# Autodesk Inventor assembly: 15102898-16-A-0200
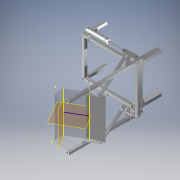
[picture p0: Inventor's stored thumbnail of the model, 180x180]
Saved by Autodesk Inventor 2017 (Build 210142000, 142)
## iProperties
Created: 2016-09-26
Part Number: 15102898-16-A-0200
Document SubType Name: Assembly
Designer: gus
Mass: 7782.67 g
Surface Area: 18020.1 cm^2
Volume: 2883.8 cm^3
Density: 2.69875 g/cm^3
Author: gus
## Documents named in this file (27)
- \\Mac\Home\Desktop\bunnybots 2016\15102898-16-Bunnybot-CAD\Bunnybot-To_be_renamed\15102898-16-A-0000\15102898-16-A-0200\15102898-16-A-0200.iam
- \\Mac\Home\Desktop\bunnybots 2016\15102898-16-Bunnybot-CAD\Bunnybot-To_be_renamed\15102898-16-A-0000\15102898-16-A-0200\15102898-16-P-0201.ipt
- \\Mac\Home\Desktop\bunnybots 2016\15102898-16-Bunnybot-CAD\Bunnybot-To_be_renamed\15102898-16-A-0000\15102898-16-A-0200\Imported Components\217-2732.20121205.ipt
- \\Mac\Home\Desktop\bunnybots 2016\15102898-16-Bunnybot-CAD\Bunnybot-To_be_renamed\15102898-16-A-0000\15102898-16-A-0200\15102898-16-P-0201_MIR.ipt
- \\Mac\Home\Desktop\bunnybots 2016\15102898-16-Bunnybot-CAD\Bunnybot-To_be_renamed\15102898-16-A-0000\15102898-16-A-0200\Imported Components\217-2732.20121205_MIR.ipt
- \\Mac\Home\Desktop\bunnybots 2016\15102898-16-Bunnybot-CAD\Bunnybot-To_be_renamed\15102898-16-A-0000\15102898-16-A-0200\15102898-16-P-0203.ipt
- \\Mac\Home\Desktop\bunnybots 2016\15102898-16-Bunnybot-CAD\Bunnybot-To_be_renamed\15102898-16-A-0000\15102898-16-A-0200\15102898-16-A-0205.ipt
- \\Mac\Home\Desktop\bunnybots 2016\15102898-16-Bunnybot-CAD\Bunnybot-To_be_renamed\15102898-16-A-0000\15102898-16-A-0200\AIS2015\175-DPEE5(F,D-231-1).iam
- \\Mac\Home\Desktop\bunnybots 2016\15102898-16-Bunnybot-CAD\Bunnybot-To_be_renamed\15102898-16-A-0000\15102898-16-A-0200\15102898-16-A-0204.iam
- \\Mac\Home\Desktop\bunnybots 2016\15102898-16-Bunnybot-CAD\Bunnybot-To_be_renamed\15102898-16-A-0000\15102898-16-A-0200\15102898-16-P-0205.ipt
- \\Mac\Home\Desktop\bunnybots 2016\15102898-16-Bunnybot-CAD\Bunnybot-To_be_renamed\15102898-16-A-0000\15102898-16-A-0200\Imported Components\91257A636_HIGH-STRENGTH GRADE 8 STEEL CAP SCREW.ipt
- \\Mac\Home\Desktop\bunnybots 2016\15102898-16-Bunnybot-CAD\Bunnybot-To_be_renamed\15102898-16-A-0000\15102898-16-A-0200\Imported Components\97135A230_GRADE 8 STEEL NYLON-INSERT LOCKNUT.ipt
- \\Mac\Home\Desktop\bunnybots 2016\15102898-16-Bunnybot-CAD\Bunnybot-To_be_renamed\15102898-16-A-0000\15102898-16-A-0200\15102898-16-P-0206.ipt
- \\Mac\Home\Desktop\bunnybots 2016\15102898-16-Bunnybot-CAD\Bunnybot-To_be_renamed\15102898-16-A-0000\15102898-16-A-0200\15102898-16-P-0207.ipt
- \\Mac\Home\Desktop\bunnybots 2016\15102898-16-Bunnybot-CAD\Bunnybot-To_be_renamed\15102898-16-A-0000\15102898-16-A-0200\15102898-16-P-0208.ipt
- \\Mac\Home\Desktop\bunnybots 2016\15102898-16-Bunnybot-CAD\Bunnybot-To_be_renamed\15102898-16-A-0000\15102898-16-A-0200\15102898-16-P-0209.ipt
- \\Mac\Home\Desktop\bunnybots 2016\15102898-16-Bunnybot-CAD\Bunnybot-To_be_renamed\15102898-16-A-0000\15102898-16-A-0200\15102898-16-P-0210.ipt
- \\Mac\Home\Desktop\bunnybots 2016\15102898-16-Bunnybot-CAD\Bunnybot-To_be_renamed\15102898-16-A-0000\15102898-16-A-0200\15102898-16-P-0211.ipt
- \\Mac\Home\Desktop\bunnybots 2016\15102898-16-Bunnybot-CAD\Bunnybot-To_be_renamed\15102898-16-A-0000\15102898-16-A-0200\15102898-16-P-0212.ipt
- \\Mac\Home\Desktop\bunnybots 2016\15102898-16-Bunnybot-CAD\Bunnybot-To_be_renamed\15102898-16-A-0000\15102898-16-A-0200\15102898-16-P-0213.ipt
- \\Mac\Home\Desktop\bunnybots 2016\15102898-16-Bunnybot-CAD\Bunnybot-To_be_renamed\15102898-16-A-0000\15102898-16-A-0200\15102898-16-P-0214.ipt
- \\Mac\Home\Desktop\bunnybots 2016\15102898-16-Bunnybot-CAD\Bunnybot-To_be_renamed\15102898-16-A-0000\15102898-16-A-0200\15102898-16-P-0215.ipt
- \\Mac\Home\Desktop\bunnybots 2016\15102898-16-Bunnybot-CAD\Bunnybot-To_be_renamed\15102898-16-A-0000\15102898-16-A-0200\15102898-16-P-0216.ipt
- \\Mac\Home\Desktop\bunnybots 2016\15102898-16-Bunnybot-CAD\Bunnybot-To_be_renamed\15102898-16-A-0000\15102898-16-A-0200\15102898-16-P-0217.ipt
- \\Mac\Home\Desktop\bunnybots 2016\15102898-16-Bunnybot-CAD\Bunnybot-To_be_renamed\15102898-16-A-0000\15102898-16-A-0200\15102898-16-P-0218.ipt
- \\Mac\Home\Desktop\bunnybots 2016\15102898-16-Bunnybot-CAD\Bunnybot-To_be_renamed\15102898-16-A-0000\15102898-16-A-0200\Imported Components\1556A170_BRACKET.ipt
- \\Mac\Home\Desktop\bunnybots 2016\15102898-16-Bunnybot-CAD\Bunnybot-To_be_renamed\15102898-16-A-0000\15102898-16-A-0200\15102898-16-P-0205_CPY.ipt
## Components (51 placed, 26 different names)
1. 15102898-16-P-0201:1 — Mate:1, Mate:4, Mate:5, Flush:9, Flush:10, Mate:14, Mate:32, Mate:42, Flush:34, Flush:35, Flush:36, Flush:56, Mate:83, Flush:91, Mate:86, Flush:94
2. 217-2732.20121205:1 — Mate:1, Mate:4, Mate:5, Cylindrical:6, Mate:22
3. 15102898-16-P-0201_MIR:1 — Flush:3, Mate:6, Mate:8, Flush:24, Mate:31, Mate:41, Flush:33, Flush:37, Mate:64, Mate:81, Flush:90, Mate:85, Flush:92, Flush:93
4. 217-2732.20121205_MIR:1 — Flush:3, Mate:6, Mate:8, Cylindrical:7, Mate:27
5. 15102898-16-P-0203:1 — Cylindrical:5, Mate:17, Mate:20, Mate:21, Cylindrical:6, Flush:40, Mate:47, Flush:59, Flush:61
6. 15102898-16-A-0205:1 — Flush:9, Flush:10, Mate:14, Mate:16, Flush:22, Flush:23, Flush:53, Flush:54, Flush:83, Flush:86, Mate:74, Flush:87, Mate:75
7. 175-DPEE5(F,D-231-1):1 [sub-assembly] — Mate:16, Cylindrical:4
8. 15102898-16-A-0204:1 [sub-assembly] — Cylindrical:4, Cylindrical:5, Mate:17
9. 15102898-16-P-0205:1 — Cylindrical:12, Mate:33, Mate:34, Mate:37, Flush:41, Mate:51, Mate:56, Flush:60
10. 15102898-16-P-0205:2 — Flush:21, Mate:26, Mate:27, Flush:42
11. 15102898-16-P-0205:3 — Flush:21, Cylindrical:13, Mate:30, Flush:51, Flush:71, Mate:62
12. 15102898-16-P-0205:4 — Mate:20, Mate:21, Mate:22, Flush:40, Flush:41
13. 15102898-16-P-0203:2 — Cylindrical:7, Mate:26, Cylindrical:9, Mate:29, Flush:42, Flush:51
14. 15102898-16-A-0205:2 — Flush:22, Flush:23, Flush:24, Flush:52, Flush:77, Mate:67, Flush:88, Mate:77, Mate:79, Flush:89
15. 175-DPEE5(F,D-231-1):2 [sub-assembly]
16. 15102898-16-A-0204:2 [sub-assembly] — Cylindrical:9, Mate:29
17. 91257A636_HIGH-STRENGTH GRADE 8 STEEL CAP SCREW:1 — Cylindrical:10, Cylindrical:13, Mate:30
18. 91257A636_HIGH-STRENGTH GRADE 8 STEEL CAP SCREW:2 — Cylindrical:11, Cylindrical:12, Mate:33, Mate:47
19. 97135A230_GRADE 8 STEEL NYLON-INSERT LOCKNUT:1 — Cylindrical:10, Mate:31
20. 97135A230_GRADE 8 STEEL NYLON-INSERT LOCKNUT:2 — Cylindrical:11, Mate:32
21. 15102898-16-P-0206:1 — Mate:34, Mate:35, Flush:27, Flush:28, Mate:36, Mate:38, Flush:31, Mate:39, Flush:63, Flush:69
22. 15102898-16-P-0207:1 — Mate:35, Flush:27, Flush:68, Flush:69
23. 15102898-16-P-0207:2 — Flush:28, Mate:36, Mate:37, Mate:51
24. 15102898-16-P-0208:1 — Mate:38, Flush:31, Flush:62, Flush:63
25. 15102898-16-P-0208:2 — Mate:39, Flush:70, Mate:60
26. 15102898-16-P-0209:1 — Mate:41, Flush:33, Mate:42, Flush:34, Mate:43, Mate:44, Mate:45
27. 15102898-16-P-0210:1 — Flush:35, Flush:36, Mate:43
28. 15102898-16-P-0210:2 — Mate:44, Flush:37, Mate:45
29. 15102898-16-P-0211:1 — Flush:52, Flush:53, Flush:54, Mate:52, Flush:55, Flush:76, Mate:68, Mate:71, Mate:73, Mate:84, Flush:95
30. 15102898-16-P-0212:1 — Mate:52, Flush:55, Cylindrical:16, Flush:56, Mate:54, Flush:81
31. 15102898-16-P-0213:1 — Cylindrical:15, Mate:55, Flush:57, Flush:58, Mate:57, Mate:58
32. 15102898-16-P-0214:1 — Cylindrical:15, Cylindrical:16, Mate:54, Mate:58, Flush:78, Flush:79
33. 15102898-16-P-0215:1 — Mate:55, Flush:57, Flush:58, Mate:63, Flush:74, Flush:75
34. 15102898-16-P-0216:1 — Flush:59, Mate:56, Flush:60, Flush:61, Flush:62, Mate:57, Flush:66, Flush:67, Flush:72, Mate:61
35. 15102898-16-P-0216:2 — Flush:66, Flush:67, Flush:68, Flush:70, Mate:60, Flush:71, Flush:73, Mate:62
36. 15102898-16-P-0217:1 — Flush:72, Mate:61, Flush:73
37. 15102898-16-P-0213:2 — Mate:63, Flush:74, Flush:75
38. 15102898-16-P-0214:2 — Flush:78, Flush:79, Mate:66
39. 15102898-16-P-0212:2 — Mate:65, Flush:80, Flush:81, Mate:66
40. 15102898-16-P-0211:2 — Flush:76, Mate:64, Flush:77, Mate:65, Flush:80, Flush:82, Mate:70, Mate:78, Mate:82
41. 15102898-16-P-0218:1 — Flush:82, Mate:67, Mate:68, Flush:83, Flush:84, Mate:69, Flush:85, Mate:72, Mate:76, Mate:80
42. 1556A170_BRACKET:1 — Flush:84, Mate:69, Mate:70
43. 1556A170_BRACKET:2 — Flush:85, Mate:71, Mate:72
44. 1556A170_BRACKET:3 — Flush:86, Mate:73, Mate:74
45. 1556A170_BRACKET:4 — Flush:87, Mate:75, Mate:76
46. 1556A170_BRACKET:5 — Flush:88, Mate:77, Mate:78
47. 1556A170_BRACKET:6 — Mate:79, Flush:89, Mate:80
48. 1556A170_BRACKET:7 — Mate:81, Mate:82, Flush:90
49. 1556A170_BRACKET:8 — Mate:83, Mate:84, Flush:91
50. 15102898-16-P-0205_CPY:1 — Mate:85, Flush:92, Flush:93
51. 15102898-16-P-0205_CPY:2 — Mate:86, Flush:94, Flush:95
## Relationships (138: Mate 65, Flush 61, CylindricalJoint 12)
- Mate:1: 15102898-16-P-0201:1 ↔ 217-2732.20121205:1
- Mate:4: 15102898-16-P-0201:1 ↔ 217-2732.20121205:1
- Mate:5: 15102898-16-P-0201:1 ↔ 217-2732.20121205:1
- Flush:3: 15102898-16-P-0201_MIR:1 ↔ 217-2732.20121205_MIR:1
- Mate:6: 15102898-16-P-0201_MIR:1 ↔ 217-2732.20121205_MIR:1
- Mate:8: 15102898-16-P-0201_MIR:1 ↔ 217-2732.20121205_MIR:1
- Flush:9: 15102898-16-P-0201:1 ↔ 15102898-16-A-0205:1
- Flush:10: 15102898-16-P-0201:1 ↔ 15102898-16-A-0205:1
- Mate:14 (467.995 mm): 15102898-16-P-0201:1 ↔ 15102898-16-A-0205:1
- Mate:16: 15102898-16-A-0205:1 ↔ 175-DPEE5(F,D-231-1):1
- Cylindrical:4: 175-DPEE5(F,D-231-1):1 ↔ 15102898-16-A-0204:1
- Cylindrical:5: 15102898-16-P-0203:1 ↔ 15102898-16-A-0204:1
- Mate:17: 15102898-16-P-0203:1 ↔ 15102898-16-A-0204:1
- Mate:20: 15102898-16-P-0203:1 ↔ 15102898-16-P-0205:4
- Mate:21: 15102898-16-P-0203:1 ↔ 15102898-16-P-0205:4
- Cylindrical:6: 217-2732.20121205:1 ↔ 15102898-16-P-0203:1
- Mate:22 (6.35 mm): 217-2732.20121205:1 ↔ 15102898-16-P-0205:4
- Flush:21: 15102898-16-P-0205:2 ↔ 15102898-16-P-0205:3
- Cylindrical:7: 217-2732.20121205_MIR:1 ↔ 15102898-16-P-0203:2
- Mate:26: 15102898-16-P-0205:2 ↔ 15102898-16-P-0203:2
- Mate:27 (6.35 mm): 217-2732.20121205_MIR:1 ↔ 15102898-16-P-0205:2
- [Mate]: 15102898-16-A-0205:2 ↔ 175-DPEE5(F,D-231-1):2
- [CylindricalJoint]: 175-DPEE5(F,D-231-1):2 ↔ 15102898-16-A-0204:2
- Flush:22: 15102898-16-A-0205:1 ↔ 15102898-16-A-0205:2
- Flush:23: 15102898-16-A-0205:1 ↔ 15102898-16-A-0205:2
- Flush:24: 15102898-16-P-0201_MIR:1 ↔ 15102898-16-A-0205:2
- Cylindrical:9: 15102898-16-P-0203:2 ↔ 15102898-16-A-0204:2
- Mate:29: 15102898-16-P-0203:2 ↔ 15102898-16-A-0204:2
- Cylindrical:10: 91257A636_HIGH-STRENGTH GRADE 8 STEEL CAP SCREW:1 ↔ 97135A230_GRADE 8 STEEL NYLON-INSERT LOCKNUT:1
- Cylindrical:11: 91257A636_HIGH-STRENGTH GRADE 8 STEEL CAP SCREW:2 ↔ 97135A230_GRADE 8 STEEL NYLON-INSERT LOCKNUT:2
- Cylindrical:12: 15102898-16-P-0205:1 ↔ 91257A636_HIGH-STRENGTH GRADE 8 STEEL CAP SCREW:2
- Cylindrical:13: 15102898-16-P-0205:3 ↔ 91257A636_HIGH-STRENGTH GRADE 8 STEEL CAP SCREW:1
- Mate:30: 15102898-16-P-0205:3 ↔ 91257A636_HIGH-STRENGTH GRADE 8 STEEL CAP SCREW:1
- Mate:31: 15102898-16-P-0201_MIR:1 ↔ 97135A230_GRADE 8 STEEL NYLON-INSERT LOCKNUT:1
- Mate:32: 15102898-16-P-0201:1 ↔ 97135A230_GRADE 8 STEEL NYLON-INSERT LOCKNUT:2
- Mate:33: 15102898-16-P-0205:1 ↔ 91257A636_HIGH-STRENGTH GRADE 8 STEEL CAP SCREW:2
- Mate:34: 15102898-16-P-0205:1 ↔ 15102898-16-P-0206:1
- Mate:35: 15102898-16-P-0206:1 ↔ 15102898-16-P-0207:1
- Flush:27: 15102898-16-P-0206:1 ↔ 15102898-16-P-0207:1
- Flush:28: 15102898-16-P-0206:1 ↔ 15102898-16-P-0207:2
- Mate:36: 15102898-16-P-0206:1 ↔ 15102898-16-P-0207:2
- Mate:37: 15102898-16-P-0205:1 ↔ 15102898-16-P-0207:2
- Mate:38: 15102898-16-P-0206:1 ↔ 15102898-16-P-0208:1
- Flush:31: 15102898-16-P-0206:1 ↔ 15102898-16-P-0208:1
- Mate:39: 15102898-16-P-0206:1 ↔ 15102898-16-P-0208:2
- Mate:41: 15102898-16-P-0201_MIR:1 ↔ 15102898-16-P-0209:1
- Flush:33: 15102898-16-P-0201_MIR:1 ↔ 15102898-16-P-0209:1
- Mate:42: 15102898-16-P-0201:1 ↔ 15102898-16-P-0209:1
- Flush:34 (38.1 mm): 15102898-16-P-0201:1 ↔ 15102898-16-P-0209:1
- Flush:35: 15102898-16-P-0201:1 ↔ 15102898-16-P-0210:1
- Flush:36: 15102898-16-P-0201:1 ↔ 15102898-16-P-0210:1
- Mate:43: 15102898-16-P-0209:1 ↔ 15102898-16-P-0210:1
- Mate:44: 15102898-16-P-0209:1 ↔ 15102898-16-P-0210:2
- Flush:37: 15102898-16-P-0201_MIR:1 ↔ 15102898-16-P-0210:2
- Mate:45: 15102898-16-P-0209:1 ↔ 15102898-16-P-0210:2
- Flush:40: 15102898-16-P-0203:1 ↔ 15102898-16-P-0205:4
- Mate:47: 15102898-16-P-0203:1 ↔ 91257A636_HIGH-STRENGTH GRADE 8 STEEL CAP SCREW:2
- Flush:41: 15102898-16-P-0205:1 ↔ 15102898-16-P-0205:4
- Flush:42: 15102898-16-P-0205:2 ↔ 15102898-16-P-0203:2
- Flush:51: 15102898-16-P-0205:3 ↔ 15102898-16-P-0203:2
- Mate:51: 15102898-16-P-0205:1 ↔ 15102898-16-P-0207:2
- Flush:52: 15102898-16-A-0205:2 ↔ 15102898-16-P-0211:1
- Flush:53: 15102898-16-A-0205:1 ↔ 15102898-16-P-0211:1
- Flush:54: 15102898-16-A-0205:1 ↔ 15102898-16-P-0211:1
- Mate:52: 15102898-16-P-0211:1 ↔ 15102898-16-P-0212:1
- Flush:55: 15102898-16-P-0211:1 ↔ 15102898-16-P-0212:1
- Cylindrical:15: 15102898-16-P-0213:1 ↔ 15102898-16-P-0214:1
- Cylindrical:16: 15102898-16-P-0212:1 ↔ 15102898-16-P-0214:1
- Flush:56 (105.7148 mm): 15102898-16-P-0201:1 ↔ 15102898-16-P-0212:1
- Mate:54: 15102898-16-P-0212:1 ↔ 15102898-16-P-0214:1
- Mate:55: 15102898-16-P-0213:1 ↔ 15102898-16-P-0215:1
- Flush:57: 15102898-16-P-0213:1 ↔ 15102898-16-P-0215:1
- Flush:58: 15102898-16-P-0213:1 ↔ 15102898-16-P-0215:1
- Flush:59: 15102898-16-P-0203:1 ↔ 15102898-16-P-0216:1
- Mate:56: 15102898-16-P-0205:1 ↔ 15102898-16-P-0216:1
- Flush:60: 15102898-16-P-0205:1 ↔ 15102898-16-P-0216:1
- Flush:61: 15102898-16-P-0203:1 ↔ 15102898-16-P-0216:1
- Flush:62: 15102898-16-P-0208:1 ↔ 15102898-16-P-0216:1
- Flush:63: 15102898-16-P-0206:1 ↔ 15102898-16-P-0208:1
- Mate:57: 15102898-16-P-0213:1 ↔ 15102898-16-P-0216:1
- Mate:58: 15102898-16-P-0213:1 ↔ 15102898-16-P-0214:1
- Flush:66: 15102898-16-P-0216:1 ↔ 15102898-16-P-0216:2
- Flush:67: 15102898-16-P-0216:1 ↔ 15102898-16-P-0216:2
- Flush:68: 15102898-16-P-0207:1 ↔ 15102898-16-P-0216:2
- Flush:69: 15102898-16-P-0206:1 ↔ 15102898-16-P-0207:1
- Flush:70: 15102898-16-P-0208:2 ↔ 15102898-16-P-0216:2
- Mate:60: 15102898-16-P-0208:2 ↔ 15102898-16-P-0216:2
- Flush:71: 15102898-16-P-0205:3 ↔ 15102898-16-P-0216:2
- Flush:72: 15102898-16-P-0216:1 ↔ 15102898-16-P-0217:1
- Mate:61: 15102898-16-P-0216:1 ↔ 15102898-16-P-0217:1
- Flush:73: 15102898-16-P-0216:2 ↔ 15102898-16-P-0217:1
- Mate:62: 15102898-16-P-0205:3 ↔ 15102898-16-P-0216:2
- Mate:63: 15102898-16-P-0215:1 ↔ 15102898-16-P-0213:2
- Flush:74: 15102898-16-P-0215:1 ↔ 15102898-16-P-0213:2
- Flush:75: 15102898-16-P-0215:1 ↔ 15102898-16-P-0213:2
- Flush:76: 15102898-16-P-0211:1 ↔ 15102898-16-P-0211:2
- Mate:64: 15102898-16-P-0201_MIR:1 ↔ 15102898-16-P-0211:2
- Flush:77: 15102898-16-A-0205:2 ↔ 15102898-16-P-0211:2
- Flush:78: 15102898-16-P-0214:1 ↔ 15102898-16-P-0214:2
- Flush:79: 15102898-16-P-0214:1 ↔ 15102898-16-P-0214:2
- Mate:65: 15102898-16-P-0212:2 ↔ 15102898-16-P-0211:2
- Flush:80: 15102898-16-P-0212:2 ↔ 15102898-16-P-0211:2
- Flush:81: 15102898-16-P-0212:1 ↔ 15102898-16-P-0212:2
- Mate:66: 15102898-16-P-0214:2 ↔ 15102898-16-P-0212:2
- Flush:82: 15102898-16-P-0211:2 ↔ 15102898-16-P-0218:1
- Mate:67: 15102898-16-A-0205:2 ↔ 15102898-16-P-0218:1
- Mate:68: 15102898-16-P-0211:1 ↔ 15102898-16-P-0218:1
- Flush:83: 15102898-16-A-0205:1 ↔ 15102898-16-P-0218:1
- Flush:84: 15102898-16-P-0218:1 ↔ 1556A170_BRACKET:1
- Mate:69: 15102898-16-P-0218:1 ↔ 1556A170_BRACKET:1
- Mate:70: 15102898-16-P-0211:2 ↔ 1556A170_BRACKET:1
- Flush:85: 15102898-16-P-0218:1 ↔ 1556A170_BRACKET:2
- Mate:71: 15102898-16-P-0211:1 ↔ 1556A170_BRACKET:2
- Mate:72: 15102898-16-P-0218:1 ↔ 1556A170_BRACKET:2
- Flush:86: 15102898-16-A-0205:1 ↔ 1556A170_BRACKET:3
- Mate:73: 15102898-16-P-0211:1 ↔ 1556A170_BRACKET:3
- Mate:74: 15102898-16-A-0205:1 ↔ 1556A170_BRACKET:3
- Flush:87: 15102898-16-A-0205:1 ↔ 1556A170_BRACKET:4
- Mate:75: 15102898-16-A-0205:1 ↔ 1556A170_BRACKET:4
- Mate:76: 15102898-16-P-0218:1 ↔ 1556A170_BRACKET:4
- Flush:88: 15102898-16-A-0205:2 ↔ 1556A170_BRACKET:5
- Mate:77: 15102898-16-A-0205:2 ↔ 1556A170_BRACKET:5
- Mate:78: 15102898-16-P-0211:2 ↔ 1556A170_BRACKET:5
- Mate:79: 15102898-16-A-0205:2 ↔ 1556A170_BRACKET:6
- Flush:89: 15102898-16-A-0205:2 ↔ 1556A170_BRACKET:6
- Mate:80: 15102898-16-P-0218:1 ↔ 1556A170_BRACKET:6
- Mate:81: 15102898-16-P-0201_MIR:1 ↔ 1556A170_BRACKET:7
- Mate:82: 15102898-16-P-0211:2 ↔ 1556A170_BRACKET:7
- Flush:90: 15102898-16-P-0201_MIR:1 ↔ 1556A170_BRACKET:7
- Mate:83: 15102898-16-P-0201:1 ↔ 1556A170_BRACKET:8
- Mate:84: 15102898-16-P-0211:1 ↔ 1556A170_BRACKET:8
- Flush:91: 15102898-16-P-0201:1 ↔ 1556A170_BRACKET:8
- Mate:85: 15102898-16-P-0201_MIR:1 ↔ 15102898-16-P-0205_CPY:1
- Flush:92: 15102898-16-P-0201_MIR:1 ↔ 15102898-16-P-0205_CPY:1
- Flush:93: 15102898-16-P-0201_MIR:1 ↔ 15102898-16-P-0205_CPY:1
- Mate:86: 15102898-16-P-0201:1 ↔ 15102898-16-P-0205_CPY:2
- Flush:94: 15102898-16-P-0201:1 ↔ 15102898-16-P-0205_CPY:2
- Flush:95: 15102898-16-P-0211:1 ↔ 15102898-16-P-0205_CPY:2
## Named parameters: d114_d59 = 0 mm, d115_d66 = 0 deg, d116_d67 = 101.6 mm, d117_d68 = 101.55448 mm, d118_d69 = -25.4 mm
